# Autodesk Inventor assembly: stackedSpoolV02
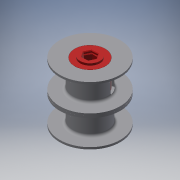
[picture p0: Inventor's stored thumbnail of the model, 180x180]
Saved by Autodesk Inventor 2019.3 (Build 233278000, 278)
## iProperties
Created: 2019-03-05
Part Number: stackedSpoolV02
Document SubType Name: Assembly
Designer: steele
Author: steele
## Documents named in this file (5)
- C:\git\CAD-Development\robSteele\RevRoboticsExtrusionAttachements\stackedSpoolV02.iam
- c:\git\CAD-MfgResources\McMaster-Carr\BrassHeatSetInsertForPlastic\6-32 0_281 94459A290_BRASS HEAT-SET INSERT FOR PLASTIC.ipt
- C:\git\CAD-Development\robSteele\RevRoboticsExtrusionAttachements\spacerForEndV05.ipt
- C:\git\CAD-Development\robSteele\RevRoboticsExtrusionAttachements\spoolV05.ipt
- C:\git\CAD-Development\robSteele\RevRoboticsExtrusionAttachements\customWasher.ipt
## Components (9 placed, 4 different names)
1. spoolV05:1 — Insert:8, Insert:9
2. spoolV05:2 — Insert:7, Insert:9, Insert:10, Insert:11
3. spacerForEndV05:2 — Insert:10
4. 6-32 0_281 94459A290_BRASS HEAT-SET INSERT FOR PLASTIC:1 — Insert:7
5. 6-32 0_281 94459A290_BRASS HEAT-SET INSERT FOR PLASTIC:2 — Insert:8
6. customWasher:1 — Insert:11, Insert:12, Flush:1
7. customWasher:2 — Insert:12, Flush:1, Insert:13
8. customWasher:3 — Insert:13, Insert:14, Flush:2
9. customWasher:4 — Insert:14, Flush:2
## Relationships (10: Insert 8, Flush 2)
- Insert:7: spoolV05:2 ↔ 6-32 0_281 94459A290_BRASS HEAT-SET INSERT FOR PLASTIC:1
- Insert:8: spoolV05:1 ↔ 6-32 0_281 94459A290_BRASS HEAT-SET INSERT FOR PLASTIC:2
- Insert:9: spoolV05:1 ↔ spoolV05:2
- Insert:10: spoolV05:2 ↔ spacerForEndV05:2
- Insert:11: spoolV05:2 ↔ customWasher:1
- Insert:12: customWasher:1 ↔ customWasher:2
- Flush:1: customWasher:1 ↔ customWasher:2
- Insert:13: customWasher:2 ↔ customWasher:3
- Insert:14: customWasher:3 ↔ customWasher:4
- Flush:2: customWasher:3 ↔ customWasher:4
